# Autodesk Inventor assembly: クランク
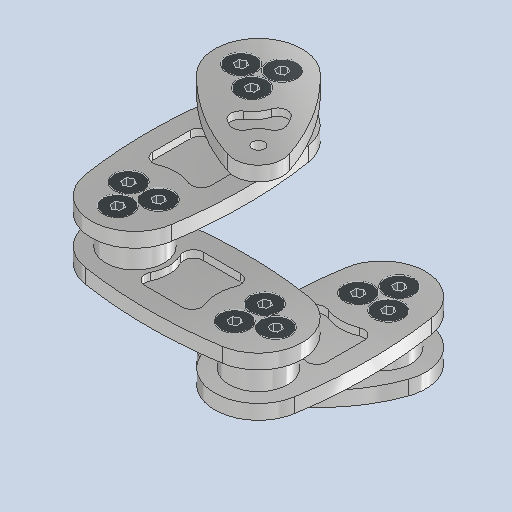
[picture p0: Inventor's stored thumbnail of the model, 512x512]
Saved by Autodesk Inventor 2023 (Build 270158000, 158)
## iProperties
Created: 2022-01-08
Part Number: クランク
Document SubType Name: Assembly
Designer: acps
Author: acps
## Documents named in this file (6)
- C:\Users\muzho\Documents\srdc\srdc_2\脚\クランク.iam
- C:\Users\muzho\Documents\srdc\srdc_2\カム\カム3.ipt
- C:\Users\muzho\Documents\srdc\srdc_2\クランク\クランク_前.ipt
- C:\Users\muzho\Documents\srdc\srdc_2\クランク\駆動節.ipt
- C:\Users\muzho\Documents\srdc\srdc_2\クランク\クランク_中間.ipt
- C:\Users\muzho\Documents\srdc\srdc_2\ねじ\m3皿ネジ10.ipt
## Components (21 placed, 5 different names)
1. カム3:1 — Mate:3, Mate:4, Insert:2, Mate:17, Mate:18, Insert:9
2. カム3:2 — Mate:5, Mate:6, Insert:3, Mate:7, Mate:8, Insert:4
3. カム3:3 — Mate:9, Mate:10, Mate:11, Mate:12, Insert:6, Insert:10
4. クランク_前:1 — Mate:17, Mate:18, Insert:9, 挿入:11, 挿入:12, 挿入:13
5. クランク_中間:1 — Mate:3, Mate:4, Insert:2, Mate:5, Mate:6, Insert:3, 挿入:20, 挿入:21, 挿入:22
6. クランク_中間:2 — Mate:7, Mate:8, Insert:4, Mate:9, Mate:10, Insert:10, 挿入:17, 挿入:18, 挿入:19
7. クランク_中間:3 — Mate:11, Mate:12, Insert:6, Mate:13, Mate:14, Insert:7, 挿入:14, 挿入:15, 挿入:16
8. カム3:4 — Mate:13, Mate:14, Insert:7, Mate:15, Mate:16, Insert:8
9. 駆動節:1 — Mate:15, Mate:16, Insert:8
10. m3皿ネジ10:1 — 挿入:11
11. m3皿ネジ10:2 — 挿入:18
12. m3皿ネジ10:3 — 挿入:16
13. m3皿ネジ10:4 — 挿入:12
14. m3皿ネジ10:5 — 挿入:20
15. m3皿ネジ10:6 — 挿入:17
16. m3皿ネジ10:7 — 挿入:19
17. m3皿ネジ10:8 — 挿入:21
18. m3皿ネジ10:9 — 挿入:14
19. m3皿ネジ10:10 — 挿入:13
20. m3皿ネジ10:11 — 挿入:15
21. m3皿ネジ10:12 — 挿入:22
## Relationships (36: Insert 20, Mate 16)
- Mate:3: カム3:1 ↔ クランク_中間:1
- Mate:4: カム3:1 ↔ クランク_中間:1
- Insert:2: カム3:1 ↔ クランク_中間:1
- Mate:5: カム3:2 ↔ クランク_中間:1
- Mate:6: カム3:2 ↔ クランク_中間:1
- Insert:3: カム3:2 ↔ クランク_中間:1
- Mate:7: カム3:2 ↔ クランク_中間:2
- Mate:8: カム3:2 ↔ クランク_中間:2
- Insert:4: カム3:2 ↔ クランク_中間:2
- Mate:9: カム3:3 ↔ クランク_中間:2
- Mate:10: カム3:3 ↔ クランク_中間:2
- Mate:11: カム3:3 ↔ クランク_中間:3
- Mate:12: カム3:3 ↔ クランク_中間:3
- Insert:6: カム3:3 ↔ クランク_中間:3
- Mate:13: クランク_中間:3 ↔ カム3:4
- Mate:14: クランク_中間:3 ↔ カム3:4
- Insert:7: クランク_中間:3 ↔ カム3:4
- Mate:15: カム3:4 ↔ 駆動節:1
- Mate:16: カム3:4 ↔ 駆動節:1
- Insert:8: カム3:4 ↔ 駆動節:1
- Mate:17: カム3:1 ↔ クランク_前:1
- Mate:18: カム3:1 ↔ クランク_前:1
- Insert:9: カム3:1 ↔ クランク_前:1
- Insert:10: カム3:3 ↔ クランク_中間:2
- 挿入:11 [Insert]: クランク_前:1 ↔ m3皿ネジ10:1
- 挿入:12 [Insert]: クランク_前:1 ↔ m3皿ネジ10:4
- 挿入:13 [Insert]: クランク_前:1 ↔ m3皿ネジ10:10
- 挿入:14 [Insert]: クランク_中間:3 ↔ m3皿ネジ10:9
- 挿入:15 [Insert]: クランク_中間:3 ↔ m3皿ネジ10:11
- 挿入:16 [Insert]: クランク_中間:3 ↔ m3皿ネジ10:3
- 挿入:17 [Insert]: クランク_中間:2 ↔ m3皿ネジ10:6
- 挿入:18 [Insert]: クランク_中間:2 ↔ m3皿ネジ10:2
- 挿入:19 [Insert]: クランク_中間:2 ↔ m3皿ネジ10:7
- 挿入:20 [Insert]: クランク_中間:1 ↔ m3皿ネジ10:5
- 挿入:21 [Insert]: クランク_中間:1 ↔ m3皿ネジ10:8
- 挿入:22 [Insert]: クランク_中間:1 ↔ m3皿ネジ10:12
